# Autodesk Inventor assembly: Turret Shooter Assembly
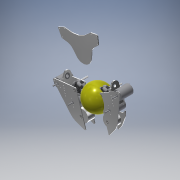
[picture p0: Inventor's stored thumbnail of the model, 180x180]
Saved by Autodesk Inventor 2019.4 (Build 234330000, 330)
## iProperties
Created: 2020-01-06
Part Number: Turret Shooter Assembly
Document SubType Name: Assembly
Designer: admin
Mass: 4067.01 g
Surface Area: 6466.54 cm^2
Volume: 4994.12 cm^3
Density: 0.814359 g/cm^3
Author: admin
## Documents named in this file (13)
- C:\Users\admin\Desktop\FRC 2020 Engineering\GitHub\7738-2020\Turret\Turret Shooter Assembly.iam
- C:\Users\admin\Desktop\FRC 2020 Engineering\GitHub\7738-2020\Turret\Omni Wheel\3_25_Omni-Directional_Wheel_217-4775.iam
- C:\Users\admin\Desktop\FRC 2020 Engineering\GitHub\7738-2020\Power Cell.ipt
- C:\Users\admin\Desktop\FRC 2020 Engineering\GitHub\7738-2020\Turret\Flywheel.ipt
- C:\Users\admin\Desktop\FRC 2020 Engineering\GitHub\7738-2020\Turret\Mini CIM\Mini_CIM_Motor_217-3371.ipt
- C:\Users\admin\Desktop\FRC 2020 Engineering\GitHub\7738-2020\CAD\Gearbox\F6800.ipt
- C:\Users\admin\Desktop\FRC 2020 Engineering\GitHub\7738-2020\Turret\Flywheel Bracket 1.ipt
- C:\Users\admin\Desktop\FRC 2020 Engineering\GitHub\7738-2020\Turret\Pivot Plate.ipt
- C:\Users\admin\Desktop\FRC 2020 Engineering\GitHub\7738-2020\CAD\Gearbox\F6804.ipt
- C:\Users\admin\Desktop\FRC 2020 Engineering\GitHub\7738-2020\Turret\Pivot Plate Idle.ipt
- C:\Users\admin\Desktop\FRC 2020 Engineering\GitHub\7738-2020\Turret\Stopper Spacers.ipt
- C:\Users\admin\Desktop\FRC 2020 Engineering\GitHub\7738-2020\Turret\Flywheel Bracket 2.ipt
- C:\Users\admin\Desktop\FRC 2020 Engineering\GitHub\7738-2020\Turret\Ball Stop.ipt
## Components (31 placed, 12 different names)
1. 3_25_Omni-Directional_Wheel_217-4775:1 [sub-assembly] — Angle:1, Mate:17, Flush:7, Flush:8, Mate:99
2. Power Cell:1 — Mate:5, Mate:6
3. Flywheel:1 — Flush:3, Flush:6, Mate:8, Flush:7, Mate:24, Mate:91, Mate:115
4. Mini_CIM_Motor_217-3371:1 — Flush:3, Mate:9, Mate:10, Mate:64
5. F6800:2 — Mate:11, Mate:12
6. Flywheel Bracket 1:1 — Mate:8, Mate:9, Mate:10, Mate:11, Mate:12, Mate:25, Mate:27, Mate:29, Mate:30, Mate:83, Mate:86, Mate:87, Mate:88, Flush:12
7. F6800:3 — Mate:24, Mate:91, Mate:100, Mate:101
8. F6800:4 — Mate:32, Mate:102, Mate:103
9. F6800:5 — Mate:25, Mate:27, Mate:99
10. Pivot Plate:1 — Mate:29, Mate:30, Flush:10, Mate:83, Flush:11
11. F6804:2 — Mate:65, Mate:66
12. 3_25_Omni-Directional_Wheel_217-4775:2 [sub-assembly] — Flush:8, Mate:95
13. Flywheel:2 — Mate:45, Mate:46, Mate:60, Mate:62
14. F6800:6 — Mate:46, Mate:53, Mate:55, Mate:62
15. F6800:7 — Mate:95, Mate:97, Mate:98, Mate:111
16. F6800:9 — Mate:45, Mate:60, Mate:94, Mate:96
17. Mini_CIM_Motor_217-3371:2 — Mate:61, Mate:63, Mate:64
18. Flywheel Bracket 1:2 — Mate:53, Mate:55, Mate:61, Mate:63, Mate:67, Mate:84, Mate:85, Flush:12, Mate:92, Mate:93, Mate:111, Mate:112, Mate:113
19. Pivot Plate Idle:1 — Mate:65, Mate:66, Mate:67, Flush:10, Mate:84, Mate:85, Flush:11
20. Stopper Spacers:1 — Mate:109, Mate:110
21. Stopper Spacers:2 — Mate:107
22. Stopper Spacers:3 — Mate:108
23. Stopper Spacers:4 — Mate:105, Mate:114
24. Stopper Spacers:5 — Mate:104
25. Stopper Spacers:6 — Mate:106
26. Mini_CIM_Motor_217-3371:3 — Mate:86, Mate:87, Mate:88
27. Flywheel Bracket 2:2 — Mate:94, Mate:96, Mate:97, Mate:98, Mate:107, Mate:108, Mate:109, Mate:110
28. Mini_CIM_Motor_217-3371:4 — Mate:92, Mate:93
29. Flywheel Bracket 2:3 — Mate:100, Mate:101, Mate:102, Mate:103, Mate:104, Mate:105, Mate:106
30. F6800:10 — Mate:112, Mate:113
31. Ball Stop:1 — Mate:114
## Relationships (66: Mate 57, Flush 8, Angle 1)
- Flush:3 (-5 mm): Flywheel:1 ↔ Mini_CIM_Motor_217-3371:1
- Mate:5: Power Cell:1
- Mate:6: Power Cell:1
- Flush:5 (103.5 mm)
- Flush:6 (-25 mm): Flywheel:1
- Mate:8: Flywheel:1 ↔ Flywheel Bracket 1:1
- Mate:9: Mini_CIM_Motor_217-3371:1 ↔ Flywheel Bracket 1:1
- Mate:10: Mini_CIM_Motor_217-3371:1 ↔ Flywheel Bracket 1:1
- Mate:11: F6800:2 ↔ Flywheel Bracket 1:1
- Mate:12 (0.2 mm): F6800:2 ↔ Flywheel Bracket 1:1
- Angle:1 (0 deg): 3_25_Omni-Directional_Wheel_217-4775:1
- Mate:17: 3_25_Omni-Directional_Wheel_217-4775:1
- Flush:7 (5.95 mm): 3_25_Omni-Directional_Wheel_217-4775:1 ↔ Flywheel:1
- Mate:24 (5 mm): Flywheel:1 ↔ F6800:3
- Mate:25: Flywheel Bracket 1:1 ↔ F6800:5
- Mate:27 (0.2 mm): Flywheel Bracket 1:1 ↔ F6800:5
- Mate:29 (0.1 mm): Flywheel Bracket 1:1 ↔ Pivot Plate:1
- Mate:30: Flywheel Bracket 1:1 ↔ Pivot Plate:1
- Mate:32: F6800:4
- Mate:45 (5 mm): Flywheel:2 ↔ F6800:9
- Mate:46 (5 mm): Flywheel:2 ↔ F6800:6
- Mate:53: F6800:6 ↔ Flywheel Bracket 1:2
- Mate:55 (0.2 mm): F6800:6 ↔ Flywheel Bracket 1:2
- Flush:8: 3_25_Omni-Directional_Wheel_217-4775:1 ↔ 3_25_Omni-Directional_Wheel_217-4775:2
- Mate:60: Flywheel:2 ↔ F6800:9
- Mate:61: Mini_CIM_Motor_217-3371:2 ↔ Flywheel Bracket 1:2
- Mate:62: Flywheel:2 ↔ F6800:6
- Mate:63: Mini_CIM_Motor_217-3371:2 ↔ Flywheel Bracket 1:2
- Mate:64 (278.846 mm): Mini_CIM_Motor_217-3371:1 ↔ Mini_CIM_Motor_217-3371:2
- Mate:65: F6804:2 ↔ Pivot Plate Idle:1
- Mate:66 (0.2 mm): F6804:2 ↔ Pivot Plate Idle:1
- Mate:67 (0.2 mm): Flywheel Bracket 1:2 ↔ Pivot Plate Idle:1
- Flush:10: Pivot Plate:1 ↔ Pivot Plate Idle:1
- Mate:83: Flywheel Bracket 1:1 ↔ Pivot Plate:1
- Mate:84: Flywheel Bracket 1:2 ↔ Pivot Plate Idle:1
- Mate:85: Flywheel Bracket 1:2 ↔ Pivot Plate Idle:1
- Mate:86: Flywheel Bracket 1:1 ↔ Mini_CIM_Motor_217-3371:3
- Mate:87: Flywheel Bracket 1:1 ↔ Mini_CIM_Motor_217-3371:3
- Mate:88: Flywheel Bracket 1:1 ↔ Mini_CIM_Motor_217-3371:3
- Mate:91: Flywheel:1 ↔ F6800:3
- Flush:11: Pivot Plate:1 ↔ Pivot Plate Idle:1
- Flush:12: Flywheel Bracket 1:1 ↔ Flywheel Bracket 1:2
- Mate:92: Flywheel Bracket 1:2 ↔ Mini_CIM_Motor_217-3371:4
- Mate:93: Flywheel Bracket 1:2 ↔ Mini_CIM_Motor_217-3371:4
- Mate:94: F6800:9 ↔ Flywheel Bracket 2:2
- Mate:95: 3_25_Omni-Directional_Wheel_217-4775:2 ↔ F6800:7
- Mate:96 (0.2 mm): F6800:9 ↔ Flywheel Bracket 2:2
- Mate:97: F6800:7 ↔ Flywheel Bracket 2:2
- Mate:98 (0.2 mm): F6800:7 ↔ Flywheel Bracket 2:2
- Mate:99: 3_25_Omni-Directional_Wheel_217-4775:1 ↔ F6800:5
- Mate:100: F6800:3 ↔ Flywheel Bracket 2:3
- Mate:101 (0.2 mm): F6800:3 ↔ Flywheel Bracket 2:3
- Mate:102: F6800:4 ↔ Flywheel Bracket 2:3
- Mate:103 (0.2 mm): F6800:4 ↔ Flywheel Bracket 2:3
- Mate:104: Stopper Spacers:5 ↔ Flywheel Bracket 2:3
- Mate:105: Stopper Spacers:4 ↔ Flywheel Bracket 2:3
- Mate:106: Stopper Spacers:6 ↔ Flywheel Bracket 2:3
- Mate:107: Stopper Spacers:2 ↔ Flywheel Bracket 2:2
- Mate:108: Stopper Spacers:3 ↔ Flywheel Bracket 2:2
- Mate:109: Stopper Spacers:1 ↔ Flywheel Bracket 2:2
- Mate:110: Stopper Spacers:1 ↔ Flywheel Bracket 2:2
- Mate:111: F6800:7 ↔ Flywheel Bracket 1:2
- Mate:112: Flywheel Bracket 1:2 ↔ F6800:10
- Mate:113 (0.2 mm): Flywheel Bracket 1:2 ↔ F6800:10
- Mate:114: Stopper Spacers:4 ↔ Ball Stop:1
- Mate:115 (104.775 mm): Flywheel:1
